# Autodesk Inventor assembly: ARM_065_IntakeDriverAssembly
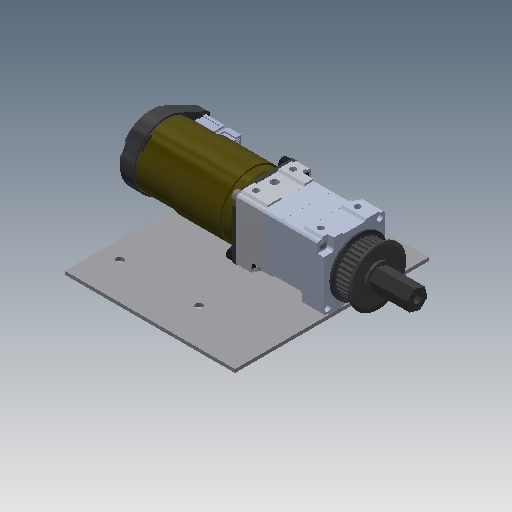
[picture p0: Inventor's stored thumbnail of the model, 512x512]
Saved by Autodesk Inventor 2018 (Build 220112000, 112)
## iProperties
Created: 2020-02-11
Part Number: ARM_065_IntakeDriverAssembly
Document SubType Name: Assembly
Designer: Sam
Author: Sam
## Documents named in this file (4)
- C:\Users\Myers.000\Documents\GrabCAD\Infinite Recharge 2020\Build season\Intake Drive\ARM_065_IntakeDriverAssembly.iam
- C:\Users\Myers.000\Documents\GrabCAD\Infinite Recharge 2020\Brainstorming\Versaplanetary\Versa+Motor.iam
- C:\Users\Myers.000\Documents\GrabCAD\Infinite Recharge 2020\Build season\Intake Drive\ARM_067_IntakeDriverMountingPlate.ipt
- C:\Users\Myers.000\Documents\GrabCAD\Infinite Recharge 2020\Build season\ARM_034_36Tx9mm3mmPitchPulley.ipt
## Components (3 placed, 3 different names)
1. Versa+Motor:1 [sub-assembly] — Flush:1, Angle:1, Insert:1, Flush:2, Mate:1
2. ARM_067_IntakeDriverMountingPlate:1 — Flush:1, Flush:2, Mate:1
3. ARM_034_36Tx9mm3mmPitchPulley:1 — Angle:1, Insert:1
## Relationships (5: Flush 2, Angle 1, Insert 1, Mate 1)
- Flush:1 (-0.0762 mm): Versa+Motor:1 ↔ ARM_067_IntakeDriverMountingPlate:1
- Angle:1 (30 deg): Versa+Motor:1 ↔ ARM_034_36Tx9mm3mmPitchPulley:1
- Insert:1: Versa+Motor:1 ↔ ARM_034_36Tx9mm3mmPitchPulley:1
- Flush:2 (-30.48 mm): Versa+Motor:1 ↔ ARM_067_IntakeDriverMountingPlate:1
- Mate:1: Versa+Motor:1 ↔ ARM_067_IntakeDriverMountingPlate:1
